# Autodesk Inventor assembly: linear bearing shroud V1
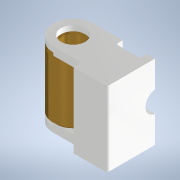
[picture p0: Inventor's stored thumbnail of the model, 180x180]
Saved by Autodesk Inventor 2020 (Build 240168000, 168)
## iProperties
Created: 2021-02-25
Part Number: linear bearing shroud V1
Document SubType Name: Assembly
Designer: AOB
Mass: 35.3529 g
Surface Area: 102.102 cm^2
Volume: 12.7073 cm^3
Density: 2.7821 g/cm^3
Author: AOB
## Documents named in this file (5)
- C:\Users\marti\Documents\Inventor\ProjectBoron\ultimate boron\linear bearing shroud V1.iam
- Y-linear bearing shroud V1.iam
- C:\Users\marti\Documents\Inventor\ProjectBoron\ultimate boron\lm8uu-graphite.ipt
- C:\Users\marti\Documents\Inventor\ProjectBoron\ultimate boron\Y-linear bearing shroud primary (2).ipt
- C:\Users\marti\Documents\Inventor\ProjectBoron\ultimate boron\Y-linear bearing shroud secondary.ipt
## Components (3 placed, 3 different names)
1. linear bearing shroud-right half V1:1 — Flush:1, Rigid:1
2. Y-linear bearing shroud primary (2):1 — Flush:1, Rigid:1, Mate:1, Mate:2
3. lm8uu-graphite:1 — Mate:1, Mate:2
## Relationships (4: Mate 2, Flush 1, WeldJoint 1)
- Flush:1: linear bearing shroud-right half V1:1 ↔ Y-linear bearing shroud primary (2):1
- Rigid:1 [WeldJoint]: linear bearing shroud-right half V1:1 ↔ Y-linear bearing shroud primary (2):1
- Mate:1: Y-linear bearing shroud primary (2):1 ↔ lm8uu-graphite:1
- Mate:2: Y-linear bearing shroud primary (2):1 ↔ lm8uu-graphite:1
